# Autodesk Inventor assembly: main_assembly
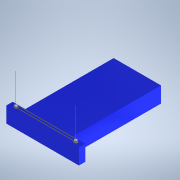
[picture p0: Inventor's stored thumbnail of the model, 180x180]
Saved by Autodesk Inventor 2020 (Build 240168000, 168)
## iProperties
Created: 2021-03-06
Part Number: main_assembly
Document SubType Name: Assembly
Designer: Harry
Author: Harry
## Documents named in this file (5)
- C:\Users\Harry\Documents\hacktheburgh\octocatch\cad\main_assembly.iam
- C:\Users\Harry\Documents\hacktheburgh\octocatch\cad\backplate.ipt
- C:\Users\Harry\Documents\hacktheburgh\octocatch\cad\dc_motor_larger.ipt
- C:\Users\Harry\Documents\hacktheburgh\octocatch\cad\belt_gear.ipt
- C:\Users\Harry\Documents\hacktheburgh\octocatch\cad\main_assembly\Design Accelerator\Synchronous Belts Transmission1.iam
## Components (6 placed, 4 different names)
1. backplate:1 — Insert:1, Insert:2
2. dc_motor_larger:1 — Insert:1, Insert:3
3. dc_motor_larger:2 — Insert:2, Insert:4
4. belt_gear:1 — Insert:3
5. belt_gear:2 — Insert:4
6. Synchronous Belts Transmission:1 [sub-assembly]
## Relationships (4: Insert 4)
- Insert:1: backplate:1 ↔ dc_motor_larger:1
- Insert:2: backplate:1 ↔ dc_motor_larger:2
- Insert:3: dc_motor_larger:1 ↔ belt_gear:1
- Insert:4: dc_motor_larger:2 ↔ belt_gear:2
